# Autodesk Inventor assembly: Ensamble eléctrico
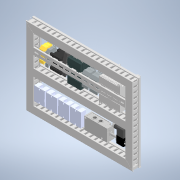
[picture p0: Inventor's stored thumbnail of the model, 180x180]
Saved by Autodesk Inventor 2021 (Build 250183000, 183)
## iProperties
Created: 2021-04-14
Part Number: Ensamble eléctrico
Document SubType Name: Assembly
Designer: Nelson
Author: Nelson
## Documents named in this file (16)
- D:\Nelson\Documentos\Inventor\Proyecto_PAI\Ensamble eléctrico.iam
- D:\Nelson\Documentos\Inventor\Proyecto_PAI\caja area de trabajo.ipt
- D:\Nelson\Documentos\Inventor\Proyecto_PAI\PLC-CP1E_N20DT1_D.iam
- D:\Nelson\Documentos\Inventor\Proyecto_PAI\FuenteDC.iam
- D:\Nelson\Documentos\Inventor\Proyecto_PAI\Rele de estado solido.ipt
- D:\Nelson\Documentos\Inventor\Proyecto_PAI\Portafusible para fusible de 2A.ipt
- D:\Nelson\Documentos\Inventor\Proyecto_PAI\Bobina_Electrovalvula.iam
- D:\Nelson\Documentos\Inventor\Proyecto_PAI\Electrovalvula-5_2.ipt
- D:\Nelson\Documentos\Inventor\Proyecto_PAI\Contactor.ipt
- D:\Nelson\Documentos\Inventor\Proyecto_PAI\Riel 35x7.5 378mm.ipt
- D:\Nelson\Documentos\Inventor\Proyecto_PAI\Bornera_AC.ipt
- D:\Nelson\Documentos\Inventor\Proyecto_PAI\Bornera_DC.ipt
- D:\Nelson\Documentos\Inventor\Proyecto_PAI\Bornera_Tierra.ipt
- D:\Nelson\Documentos\Inventor\Proyecto_PAI\Canaleta 30x30 438mm.iam
- D:\Nelson\Documentos\Inventor\Proyecto_PAI\Canaleta 30x30 378mm.iam
- D:\Nelson\Documentos\Inventor\Proyecto_PAI\Canaleta 30x30 317mm.iam
## Components (31 placed, 15 different names)
1. caja area de trabajo:1 — Mate:1, Flush:1, Mate:66, Mate:67
2. PLC-CP1E_N20DT1_D:1 [sub-assembly] — Mate:13, Mate:14, Flush:16, Mate:59
3. FuenteDC:1 [sub-assembly] — Mate:15, Mate:16, Mate:61, Mate:62
4. Rele de estado solido:1 — Flush:29, Flush:30, Flush:33
5. Portafusible para fusible de 2A:1 — Mate:17, Mate:18, Mate:62, Mate:63
6. Bobina_Electrovalvula:1 [sub-assembly] — Mate:9, Flush:13, Flush:14
7. Electrovalvula-5_2:1 — Mate:9, Flush:13, Flush:14, Flush:28
8. Contactor:1 — Mate:19, Mate:20, Mate:63, Mate:64
9. Riel 35x7.5 378mm:1 — Mate:13, Mate:14, Mate:15, Mate:16, Mate:17, Mate:18, Mate:19, Mate:20, Mate:21, Mate:22, Mate:23, Mate:24, Mate:26, Mate:27, Mate:28, Mate:29, Mate:31, Mate:32, Mate:34, Mate:35, Mate:37, Mate:38, Mate:39, Mate:40, Mate:42, Mate:43, Mate:45, Mate:46, Mate:48, Mate:49, Mate:51, Mate:52, Mate:53, Mate:54, Mate:56, Mate:57, Flush:16, Flush:20, Mate:72
10. Bornera_AC:1 — Mate:21, Mate:22, Mate:25, Mate:64
11. Bornera_AC:2 — Mate:23, Mate:24, Mate:25, Mate:65
12. Bornera_DC:1 — Mate:26, Mate:27, Mate:30, Mate:61
13. Bornera_DC:2 — Mate:28, Mate:29, Mate:30, Mate:33
14. Bornera_DC:3 — Mate:31, Mate:32, Mate:33, Mate:36
15. Bornera_DC:4 — Mate:34, Mate:35, Mate:36, Mate:60
16. Bornera_DC:5 — Mate:39, Mate:40, Mate:41, Mate:44
17. Bornera_DC:6 — Mate:42, Mate:43, Mate:44, Mate:47
18. Bornera_DC:7 — Mate:45, Mate:46, Mate:47, Mate:50
19. Bornera_DC:8 — Mate:48, Mate:49, Mate:50, Mate:59
20. Bornera_DC:9 — Mate:37, Mate:38, Mate:41, Mate:60
21. Bornera_Tierra:1 — Mate:51, Mate:52, Mate:55, Mate:65
22. Bornera_Tierra:2 — Mate:53, Mate:54, Mate:55, Mate:58
23. Bornera_Tierra:3 — Mate:56, Mate:57, Mate:58
24. Rele de estado solido:2 — Flush:30, Flush:31, Flush:33, Flush:34
25. Rele de estado solido:3 — Flush:31, Flush:32, Flush:34, Flush:35
26. Rele de estado solido:4 — Flush:32, Flush:35
27. Canaleta 30x30 438mm:1 [sub-assembly] — Mate:67, Mate:68, Flush:17, Mate:71, Flush:20
28. Canaleta 30x30 438mm:2 [sub-assembly] — Flush:18, Mate:69, Mate:70, Flush:19
29. Canaleta 30x30 378mm:1 [sub-assembly] — Flush:21, Mate:73, Flush:28, Flush:29
30. Canaleta 30x30 317mm:1 [sub-assembly] — Mate:66, Mate:68, Flush:17, Flush:18, Mate:69, Mate:72
31. Canaleta 30x30 317mm:2 [sub-assembly] — Mate:70, Flush:19, Mate:71, Flush:21, Mate:73
## Relationships (80: Mate 63, Flush 17)
- Mate:1: caja area de trabajo:1
- Flush:1: caja area de trabajo:1
- Mate:9: Bobina_Electrovalvula:1 ↔ Electrovalvula-5_2:1
- Flush:13: Bobina_Electrovalvula:1 ↔ Electrovalvula-5_2:1
- Flush:14: Bobina_Electrovalvula:1 ↔ Electrovalvula-5_2:1
- Mate:13: PLC-CP1E_N20DT1_D:1 ↔ Riel 35x7.5 378mm:1
- Mate:14: PLC-CP1E_N20DT1_D:1 ↔ Riel 35x7.5 378mm:1
- Mate:15: FuenteDC:1 ↔ Riel 35x7.5 378mm:1
- Mate:16: FuenteDC:1 ↔ Riel 35x7.5 378mm:1
- Mate:17: Portafusible para fusible de 2A:1 ↔ Riel 35x7.5 378mm:1
- Mate:18: Portafusible para fusible de 2A:1 ↔ Riel 35x7.5 378mm:1
- Mate:19: Contactor:1 ↔ Riel 35x7.5 378mm:1
- Mate:20: Contactor:1 ↔ Riel 35x7.5 378mm:1
- Mate:21: Riel 35x7.5 378mm:1 ↔ Bornera_AC:1
- Mate:22: Riel 35x7.5 378mm:1 ↔ Bornera_AC:1
- Mate:23: Riel 35x7.5 378mm:1 ↔ Bornera_AC:2
- Mate:24: Riel 35x7.5 378mm:1 ↔ Bornera_AC:2
- Mate:25: Bornera_AC:1 ↔ Bornera_AC:2
- Mate:26: Riel 35x7.5 378mm:1 ↔ Bornera_DC:1
- Mate:27: Riel 35x7.5 378mm:1 ↔ Bornera_DC:1
- Mate:28: Riel 35x7.5 378mm:1 ↔ Bornera_DC:2
- Mate:29: Riel 35x7.5 378mm:1 ↔ Bornera_DC:2
- Mate:30: Bornera_DC:1 ↔ Bornera_DC:2
- Mate:31: Riel 35x7.5 378mm:1 ↔ Bornera_DC:3
- Mate:32: Riel 35x7.5 378mm:1 ↔ Bornera_DC:3
- Mate:33: Bornera_DC:2 ↔ Bornera_DC:3
- Mate:34: Riel 35x7.5 378mm:1 ↔ Bornera_DC:4
- Mate:35: Riel 35x7.5 378mm:1 ↔ Bornera_DC:4
- Mate:36: Bornera_DC:3 ↔ Bornera_DC:4
- Mate:37: Riel 35x7.5 378mm:1 ↔ Bornera_DC:9
- Mate:38: Riel 35x7.5 378mm:1 ↔ Bornera_DC:9
- Mate:39: Riel 35x7.5 378mm:1 ↔ Bornera_DC:5
- Mate:40: Riel 35x7.5 378mm:1 ↔ Bornera_DC:5
- Mate:41: Bornera_DC:5 ↔ Bornera_DC:9
- Mate:42: Riel 35x7.5 378mm:1 ↔ Bornera_DC:6
- Mate:43: Riel 35x7.5 378mm:1 ↔ Bornera_DC:6
- Mate:44: Bornera_DC:5 ↔ Bornera_DC:6
- Mate:45: Riel 35x7.5 378mm:1 ↔ Bornera_DC:7
- Mate:46: Riel 35x7.5 378mm:1 ↔ Bornera_DC:7
- Mate:47: Bornera_DC:6 ↔ Bornera_DC:7
- Mate:48: Riel 35x7.5 378mm:1 ↔ Bornera_DC:8
- Mate:49: Riel 35x7.5 378mm:1 ↔ Bornera_DC:8
- Mate:50: Bornera_DC:7 ↔ Bornera_DC:8
- Mate:51: Riel 35x7.5 378mm:1 ↔ Bornera_Tierra:1
- Mate:52: Riel 35x7.5 378mm:1 ↔ Bornera_Tierra:1
- Mate:53: Riel 35x7.5 378mm:1 ↔ Bornera_Tierra:2
- Mate:54: Riel 35x7.5 378mm:1 ↔ Bornera_Tierra:2
- Mate:55: Bornera_Tierra:1 ↔ Bornera_Tierra:2
- Mate:56: Riel 35x7.5 378mm:1 ↔ Bornera_Tierra:3
- Mate:57: Riel 35x7.5 378mm:1 ↔ Bornera_Tierra:3
- Mate:58: Bornera_Tierra:2 ↔ Bornera_Tierra:3
- Flush:16 (24 mm): PLC-CP1E_N20DT1_D:1 ↔ Riel 35x7.5 378mm:1
- Mate:59 (7 mm): PLC-CP1E_N20DT1_D:1 ↔ Bornera_DC:8
- Mate:60 (7 mm): Bornera_DC:4 ↔ Bornera_DC:9
- Mate:61 (7 mm): FuenteDC:1 ↔ Bornera_DC:1
- Mate:62 (7 mm): FuenteDC:1 ↔ Portafusible para fusible de 2A:1
- Mate:63 (7 mm): Portafusible para fusible de 2A:1 ↔ Contactor:1
- Mate:64 (7 mm): Contactor:1 ↔ Bornera_AC:1
- Mate:65 (7 mm): Bornera_AC:2 ↔ Bornera_Tierra:1
- Mate:66: caja area de trabajo:1 ↔ Canaleta 30x30 317mm:1
- Mate:67: caja area de trabajo:1 ↔ Canaleta 30x30 438mm:1
- Mate:68: Canaleta 30x30 438mm:1 ↔ Canaleta 30x30 317mm:1
- Flush:17: Canaleta 30x30 438mm:1 ↔ Canaleta 30x30 317mm:1
- Flush:18: Canaleta 30x30 438mm:2 ↔ Canaleta 30x30 317mm:1
- Mate:69: Canaleta 30x30 438mm:2 ↔ Canaleta 30x30 317mm:1
- Mate:70: Canaleta 30x30 438mm:2 ↔ Canaleta 30x30 317mm:2
- Flush:19: Canaleta 30x30 438mm:2 ↔ Canaleta 30x30 317mm:2
- Mate:71: Canaleta 30x30 438mm:1 ↔ Canaleta 30x30 317mm:2
- Flush:20: Riel 35x7.5 378mm:1 ↔ Canaleta 30x30 438mm:1
- Mate:72: Riel 35x7.5 378mm:1 ↔ Canaleta 30x30 317mm:1
- Flush:21: Canaleta 30x30 378mm:1 ↔ Canaleta 30x30 317mm:2
- Mate:73: Canaleta 30x30 378mm:1 ↔ Canaleta 30x30 317mm:2
- Flush:28: Electrovalvula-5_2:1 ↔ Canaleta 30x30 378mm:1
- Flush:29: Rele de estado solido:1 ↔ Canaleta 30x30 378mm:1
- Flush:30: Rele de estado solido:1 ↔ Rele de estado solido:2
- Flush:31: Rele de estado solido:2 ↔ Rele de estado solido:3
- Flush:32: Rele de estado solido:3 ↔ Rele de estado solido:4
- Flush:33: Rele de estado solido:1 ↔ Rele de estado solido:2
- Flush:34: Rele de estado solido:2 ↔ Rele de estado solido:3
- Flush:35: Rele de estado solido:3 ↔ Rele de estado solido:4
